# Autodesk Inventor assembly: step driver support
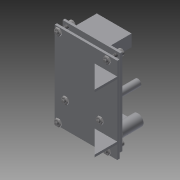
[picture p0: Inventor's stored thumbnail of the model, 180x180]
Saved by Autodesk Inventor 2015 (Build 190159000, 159)
## iProperties
Created: 2015-05-04
Part Number: step driver support
Document SubType Name: Assembly
Designer: Kuba
Author: Kuba
## Documents named in this file (6)
- C:\Users\Kuba\Dysk Google\synergia\Synergolf\model\GOLF\step driver support\step driver support.iam
- C:\Users\Kuba\Dysk Google\synergia\Synergolf\model\GOLF\step driver support\step driver.ipt
- C:\Users\Kuba\Dysk Google\synergia\Synergolf\model\GOLF\step driver support\blacha pionowa ste driver.ipt
- C:\Users\Kuba\Dysk Google\synergia\Synergolf\model\GOLF\driver\wspornik.ipt
- C:\Users\Kuba\Dysk Google\synergia\Synergolf\model\GOLF\ContentCenter\pl-PL\DIN 912\DIN 912 - M3 x 0,5 x 12 x 10,75.ipt
- C:\Users\Kuba\Dysk Google\synergia\Synergolf\model\GOLF\ContentCenter\pl-PL\DIN 439-2\DIN 439 - M3 x 0,5.ipt
## Components (16 placed, 5 different names)
1. step driver:1 — Zestawiający:1, Równoległy:1, Równoległy:2, Wstaw:1, Wstaw:2, Wstaw:3, Wstaw:4, Wstaw:5, Wstaw:6
2. blacha pionowa ste driver:1 — Zestawiający:1, Równoległy:1, Równoległy:2, Zestawiający:2, Zestawiający:3, Równoległy:3, Równoległy:4, Równoległy:5, Równoległy:6, Wstaw:7, Wstaw:8, Wstaw:9, Wstaw:10, Wstaw:11, Wstaw:12
3. wspornik:1 — Zestawiający:2, Równoległy:4, Równoległy:6
4. wspornik:2 — Zestawiający:3, Równoległy:3, Równoległy:5
5. DIN 912 - zastąpiona przez DIN EN ISO 4762 M3 x 12:1 — Wstaw:1
6. DIN 912 - zastąpiona przez DIN EN ISO 4762 M3 x 12:2 — Wstaw:2
7. DIN 912 - zastąpiona przez DIN EN ISO 4762 M3 x 12:3 — Wstaw:3
8. DIN 912 - zastąpiona przez DIN EN ISO 4762 M3 x 12:4 — Wstaw:4
9. DIN 912 - zastąpiona przez DIN EN ISO 4762 M3 x 12:5 — Wstaw:5
10. DIN 912 - zastąpiona przez DIN EN ISO 4762 M3 x 12:6 — Wstaw:6
11. DIN 439-2 - zastąpiona przez DIN EN 24035/28675 M3:1 — Wstaw:7
12. DIN 439-2 - zastąpiona przez DIN EN 24035/28675 M3:2 — Wstaw:8
13. DIN 439-2 - zastąpiona przez DIN EN 24035/28675 M3:3 — Wstaw:9
14. DIN 439-2 - zastąpiona przez DIN EN 24035/28675 M3:4 — Wstaw:10
15. DIN 439-2 - zastąpiona przez DIN EN 24035/28675 M3:5 — Wstaw:11
16. DIN 439-2 - zastąpiona przez DIN EN 24035/28675 M3:6 — Wstaw:12
## Relationships (21: Insert 12, Flush 6, Mate 3)
- Zestawiający:1 [Mate]: step driver:1 ↔ blacha pionowa ste driver:1
- Równoległy:1 [Flush]: step driver:1 ↔ blacha pionowa ste driver:1
- Równoległy:2 [Flush]: step driver:1 ↔ blacha pionowa ste driver:1
- Zestawiający:2 [Mate]: blacha pionowa ste driver:1 ↔ wspornik:1
- Zestawiający:3 [Mate]: blacha pionowa ste driver:1 ↔ wspornik:2
- Równoległy:3 [Flush]: blacha pionowa ste driver:1 ↔ wspornik:2
- Równoległy:4 [Flush]: blacha pionowa ste driver:1 ↔ wspornik:1
- Równoległy:5 [Flush] (12 mm): blacha pionowa ste driver:1 ↔ wspornik:2
- Równoległy:6 [Flush] (12 mm): blacha pionowa ste driver:1 ↔ wspornik:1
- Wstaw:1 [Insert]: step driver:1 ↔ DIN 912 - zastąpiona przez DIN EN ISO 4762 M3 x 12:1
- Wstaw:2 [Insert]: step driver:1 ↔ DIN 912 - zastąpiona przez DIN EN ISO 4762 M3 x 12:2
- Wstaw:3 [Insert]: step driver:1 ↔ DIN 912 - zastąpiona przez DIN EN ISO 4762 M3 x 12:3
- Wstaw:4 [Insert]: step driver:1 ↔ DIN 912 - zastąpiona przez DIN EN ISO 4762 M3 x 12:4
- Wstaw:5 [Insert]: step driver:1 ↔ DIN 912 - zastąpiona przez DIN EN ISO 4762 M3 x 12:5
- Wstaw:6 [Insert]: step driver:1 ↔ DIN 912 - zastąpiona przez DIN EN ISO 4762 M3 x 12:6
- Wstaw:7 [Insert]: blacha pionowa ste driver:1 ↔ DIN 439-2 - zastąpiona przez DIN EN 24035/28675 M3:1
- Wstaw:8 [Insert]: blacha pionowa ste driver:1 ↔ DIN 439-2 - zastąpiona przez DIN EN 24035/28675 M3:2
- Wstaw:9 [Insert]: blacha pionowa ste driver:1 ↔ DIN 439-2 - zastąpiona przez DIN EN 24035/28675 M3:3
- Wstaw:10 [Insert]: blacha pionowa ste driver:1 ↔ DIN 439-2 - zastąpiona przez DIN EN 24035/28675 M3:4
- Wstaw:11 [Insert]: blacha pionowa ste driver:1 ↔ DIN 439-2 - zastąpiona przez DIN EN 24035/28675 M3:5
- Wstaw:12 [Insert]: blacha pionowa ste driver:1 ↔ DIN 439-2 - zastąpiona przez DIN EN 24035/28675 M3:6
